# Autodesk Inventor assembly: polus
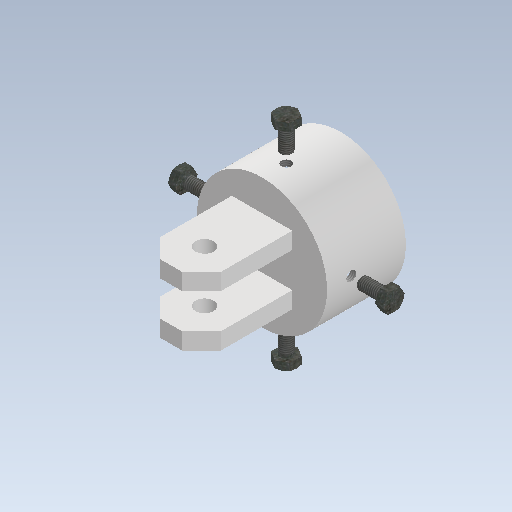
[picture p0: Inventor's stored thumbnail of the model, 512x512]
Saved by Autodesk Inventor 2021 (Build 250183000, 183)
## iProperties
Created: 2023-12-03
Part Number: polus
Document SubType Name: Assembly
Designer: vtoth
Author: vtoth
## Documents named in this file (3)
- C:\Users\ZenBook\OneDrive - Budapesti Műszaki és Gazdaságtudományi Egyetem\5_felev\CAD\hf2_v2\polus.iam
- C:\Users\ZenBook\OneDrive - Budapesti Műszaki és Gazdaságtudományi Egyetem\5_felev\CAD\hf2_v2\polus_tarto.ipt
- C:\Users\ZenBook\OneDrive - Budapesti Műszaki és Gazdaságtudományi Egyetem\Dokumentumok\Inventor\Content Center Files\R2021\en-US\ISO 4018\ISO 4018 - M8 x 16.ipt
## Components (5 placed, 2 different names)
1. polus_tarto:1 — Mate:1, Angle:1
2. ISO 4018 M8 x 16:1 — Mate:1, Angle:1
3. ISO 4018 M8 x 16:2
4. ISO 4018 M8 x 16:3
5. ISO 4018 M8 x 16:4
## Component patterns: (4 elements, first: ISO 4018 M8 x 16:1)
## Relationships (2: Mate 1, Angle 1)
- Mate:1: polus_tarto:1 ↔ ISO 4018 M8 x 16:1
- Angle:1 (0 deg): polus_tarto:1 ↔ ISO 4018 M8 x 16:1
